# Autodesk Inventor assembly: Battery holder assembly
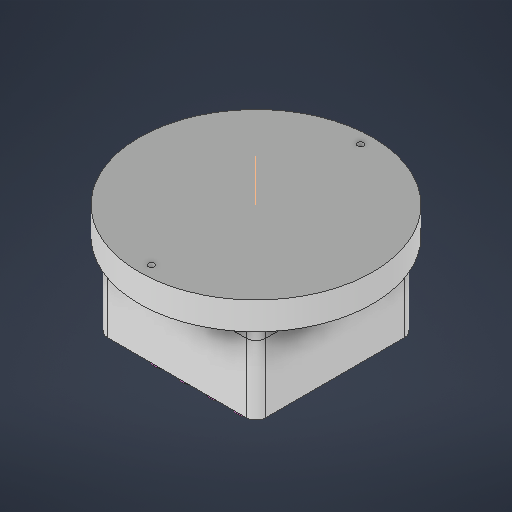
[picture p0: Inventor's stored thumbnail of the model, 512x512]
Saved by Autodesk Inventor 2025 (Build 290162000, 162)
## iProperties
Created: 2025-08-08
Part Number: Battery holder assembly
Document SubType Name: Assembly
Designer: mayhe
Author: mayhe
## Documents named in this file (5)
- C:\Users\mayhe\OneDrive\Documents\GitHub\In-situ-monitoring-of-powder-bed-fusion-additive-manufacturing\accessories\Battery Holder\Battery holder assembly.iam
- C:\Users\mayhe\OneDrive\Documents\GitHub\In-situ-monitoring-of-powder-bed-fusion-additive-manufacturing\accessories\threaded_build-plate\substrate plate With Lots of holes.ipt
- C:\Users\mayhe\OneDrive\Documents\GitHub\In-situ-monitoring-of-powder-bed-fusion-additive-manufacturing\accessories\Battery Holder\Battery Holder (Bottom).ipt
- C:\Users\mayhe\OneDrive\Documents\GitHub\In-situ-monitoring-of-powder-bed-fusion-additive-manufacturing\accessories\Battery Holder\18650(PINK).ipt
- C:\Users\mayhe\OneDrive\Documents\GitHub\In-situ-monitoring-of-powder-bed-fusion-additive-manufacturing\accessories\Battery Holder\Battery Holder (Top).ipt
## Components (21 placed, 4 different names)
1. substrate plate With Lots of holes:1 — Rotational:3, Mate:1
2. Battery Holder (Top):1 — Mate:2, Flush:1, Flush:2
3. Battery Holder (Bottom):1 — Rotational:2, Rotational:3, Mate:1, Rotational:4, Rotational:5, Rotational:6, Rotational:7, Rotational:8, Rotational:9, Rotational:10, Rotational:11, Rotational:12, Rigid:1, Rotational:13, Rigid:2, Rotational:14, Rotational:15, Rigid:3, Rotational:16, Rotational:17, Mate:2, Flush:1, Flush:2
4. 18650(PINK):1 — Rotational:2
5. 18650(PINK):2 — Rigid:2
6. 18650(PINK):3 — Rigid:3
7. 18650(PINK):4 — Rotational:15
8. 18650(PINK):5 — Rotational:14
9. 18650(PINK):6 — Rotational:7
10. 18650(PINK):7 — Rotational:9
11. 18650(PINK):8 — Rotational:10
12. 18650(PINK):9 — Rotational:11
13. 18650(PINK):10 — Rotational:12
14. 18650(PINK):11 — Rigid:1
15. 18650(PINK):12 — Rotational:13
16. 18650(PINK):13 — Rotational:8
17. 18650(PINK):14 — Rotational:16
18. 18650(PINK):15 — Rotational:6
19. 18650(PINK):16 — Rotational:5
20. 18650(PINK):17 — Rotational:4
21. 18650(PINK):18 — Rotational:17
## Relationships (23: RevoluteJoint 16, WeldJoint 3, Mate 2, Flush 2)
- Rotational:2 [RevoluteJoint]: Battery Holder (Bottom):1 ↔ 18650(PINK):1
- Rotational:3 [RevoluteJoint]: substrate plate With Lots of holes:1 ↔ Battery Holder (Bottom):1
- Mate:1: substrate plate With Lots of holes:1 ↔ Battery Holder (Bottom):1
- Rotational:4 [RevoluteJoint]: Battery Holder (Bottom):1 ↔ 18650(PINK):17
- Rotational:5 [RevoluteJoint]: Battery Holder (Bottom):1 ↔ 18650(PINK):16
- Rotational:6 [RevoluteJoint]: Battery Holder (Bottom):1 ↔ 18650(PINK):15
- Rotational:7 [RevoluteJoint]: Battery Holder (Bottom):1 ↔ 18650(PINK):6
- Rotational:8 [RevoluteJoint]: Battery Holder (Bottom):1 ↔ 18650(PINK):13
- Rotational:9 [RevoluteJoint]: Battery Holder (Bottom):1 ↔ 18650(PINK):7
- Rotational:10 [RevoluteJoint]: Battery Holder (Bottom):1 ↔ 18650(PINK):8
- Rotational:11 [RevoluteJoint]: Battery Holder (Bottom):1 ↔ 18650(PINK):9
- Rotational:12 [RevoluteJoint]: Battery Holder (Bottom):1 ↔ 18650(PINK):10
- Rigid:1 [WeldJoint]: Battery Holder (Bottom):1 ↔ 18650(PINK):11
- Rotational:13 [RevoluteJoint]: Battery Holder (Bottom):1 ↔ 18650(PINK):12
- Rigid:2 [WeldJoint]: Battery Holder (Bottom):1 ↔ 18650(PINK):2
- Rotational:14 [RevoluteJoint]: Battery Holder (Bottom):1 ↔ 18650(PINK):5
- Rotational:15 [RevoluteJoint]: Battery Holder (Bottom):1 ↔ 18650(PINK):4
- Rigid:3 [WeldJoint]: Battery Holder (Bottom):1 ↔ 18650(PINK):3
- Rotational:16 [RevoluteJoint]: Battery Holder (Bottom):1 ↔ 18650(PINK):14
- Rotational:17 [RevoluteJoint]: Battery Holder (Bottom):1 ↔ 18650(PINK):18
- Mate:2: Battery Holder (Top):1 ↔ Battery Holder (Bottom):1
- Flush:1: Battery Holder (Top):1 ↔ Battery Holder (Bottom):1
- Flush:2: Battery Holder (Top):1 ↔ Battery Holder (Bottom):1
